# Autodesk Inventor assembly: Assembly_Cube_Berrybase_CCTVLens_100mm
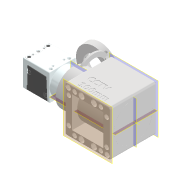
[picture p0: Inventor's stored thumbnail of the model, 180x180]
Saved by Autodesk Inventor 2022 (Build 260153000, 153)
## iProperties
Created: 2023-01-18
Part Number: Assembly_Cube_Berrybase_CCTVLens_100mm
Document SubType Name: Assembly
Designer: diederichbenedict
Author: diederichbenedict
## Documents named in this file (6)
- C:\Users\diederichbenedict\Dropbox\Dokumente\Promotion\PROJECTS\openUC2-CAD\INVENTOR\Assembly_Cube_Berrybase_CCTVLens_100mm.iam
- C:\Users\diederichbenedict\Dropbox\Dokumente\Promotion\PROJECTS\openUC2-CAD\INVENTOR\00_Basler_ace_USB3_C-Mount.ipt
- C:\Users\diederichbenedict\Dropbox\Dokumente\Promotion\PROJECTS\openUC2-CAD\INVENTOR\11_Cube_Berrybase_CCTV_100mm_Lens_Cube_half.ipt
- C:\Users\diederichbenedict\Dropbox\Dokumente\Promotion\PROJECTS\openUC2-CAD\INVENTOR\00_Berrybase_CCTVLens_100mm.ipt
- C:\Users\diederichbenedict\Dropbox\Dokumente\Promotion\PROJECTS\openUC2-CAD\INVENTOR\50_Filteradapter_Fluorescence_CCVTV_Berrybase_100mm.ipt
- C:\Users\diederichbenedict\Dropbox\Dokumente\Promotion\PROJECTS\openUC2-CAD\INVENTOR\00_CMountSpacer_CCTVLens_Daheng.ipt
## Components (6 placed, 5 different names)
1. 00_Berrybase_CCTVLens_100mm:1 — Einfügen:1, Einfügen:2, Winkel:1, Einfügen:3
2. 11_Cube_Berrybase_CCTV_100mm_Lens_Cube_half:1 — Einfügen:1, Passend:1
3. 11_Cube_Berrybase_CCTV_100mm_Lens_Cube_half:2 — Einfügen:2, Winkel:1, Passend:1
4. 00_Basler_ace_USB3_C-Mount:1 — Einfügen:3
5. 50_Filteradapter_Fluorescence_CCVTV_Berrybase_100mm:1
6. 00_CMountSpacer_CCTVLens_Daheng:1
## Relationships (5: Insert 3, Angle 1, Mate 1)
- Einfügen:1 [Insert]: 00_Berrybase_CCTVLens_100mm:1 ↔ 11_Cube_Berrybase_CCTV_100mm_Lens_Cube_half:1
- Einfügen:2 [Insert]: 00_Berrybase_CCTVLens_100mm:1 ↔ 11_Cube_Berrybase_CCTV_100mm_Lens_Cube_half:2
- Winkel:1 [Angle] (0 deg): 00_Berrybase_CCTVLens_100mm:1 ↔ 11_Cube_Berrybase_CCTV_100mm_Lens_Cube_half:2
- Passend:1 [Mate]: 11_Cube_Berrybase_CCTV_100mm_Lens_Cube_half:1 ↔ 11_Cube_Berrybase_CCTV_100mm_Lens_Cube_half:2
- Einfügen:3 [Insert]: 00_Berrybase_CCTVLens_100mm:1 ↔ 00_Basler_ace_USB3_C-Mount:1
